# Autodesk Inventor assembly: MyAssembly
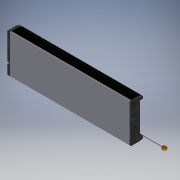
[picture p0: Inventor's stored thumbnail of the model, 180x180]
Saved by Autodesk Inventor 2016 (Build 200138000, 138)
## iProperties
Created: 2015-05-20
Part Number: MyAssembly
Document SubType Name: Assembly
Designer: Andy
Mass: 25160 g
Surface Area: 16220.2 cm^2
Volume: 5838.19 cm^3
Density: 4.30956 g/cm^3
Author: Andy
## Documents named in this file (4)
- C:\Users\jonathan\Documents\GitHub\Integrated-Tool-Suite\Inverted Pendulum\Inventor\Inverted Pendulum.iam
- C:\Users\jonathan\Documents\GitHub\Integrated-Tool-Suite\Inverted Pendulum\Inventor\Base Assembly.iam
- C:\Users\jonathan\Documents\GitHub\Integrated-Tool-Suite\Inverted Pendulum\Inventor\Track Assembly.iam
- C:\Users\jonathan\Documents\GitHub\Integrated-Tool-Suite\Inverted Pendulum\Inventor\Pendulum Assembly.iam
## Components (3 placed, 3 different names)
1. Base Assembly:1 [sub-assembly] — Angle:1, Mate:6, Mate:7
2. Track Assembly:1 [sub-assembly] — Angle:1, Mate:4, Mate:5, Mate:6, Mate:7
3. Pendulum Assembly:1 [sub-assembly] — Mate:4, Mate:5
## Relationships (5: Mate 4, Angle 1)
- Angle:1 (180 deg): Base Assembly:1 ↔ Track Assembly:1
- Mate:4: Track Assembly:1 ↔ Pendulum Assembly:1
- Mate:5 (-6 mm): Track Assembly:1 ↔ Pendulum Assembly:1
- Mate:6: Base Assembly:1 ↔ Track Assembly:1
- Mate:7: Base Assembly:1 ↔ Track Assembly:1
